# Autodesk Inventor assembly: GFRP_T2_03
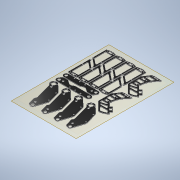
[picture p0: Inventor's stored thumbnail of the model, 180x180]
Saved by Autodesk Inventor 2022 (Build 260153000, 153)
## iProperties
Created: 2022-09-28
Part Number: GFRP_T2_03
Document SubType Name: Assembly
Designer: Masato
Author: Masato
## Documents named in this file (6)
- C:\Users\6343y\ドキュメント\Inventor\SUSTAINA-OP\Cam\GFRP_T2\OriginalMind_RD400\GFRP_T2_03.iam
- C:\Users\6343y\ドキュメント\Inventor\SUSTAINA-OP\Cam\DisposableBoard.ipt
- C:\Users\6343y\ドキュメント\Inventor\SUSTAINA-OP\LowerBody\Link\BackLink_frame.ipt
- C:\Users\6343y\ドキュメント\Inventor\SUSTAINA-OP\LowerBody\Link\FrontLink_frame.ipt
- C:\Users\6343y\ドキュメント\Inventor\SUSTAINA-OP\UpperBody\Arm\UpperArm_side_frame.ipt
- C:\Users\6343y\ドキュメント\Inventor\SUSTAINA-OP\UpperBody\Head\Head_neck_side_frame.ipt
## Components (17 placed, 5 different names)
1. DisposableBoard:1 — フラッシュ:1, フラッシュ:2, フラッシュ:3, フラッシュ:4, フラッシュ:9, フラッシュ:10, Tangent:23, Tangent:24
2. BackLink_frame:4 — メイト:21, Mate:25, Tangent:22
3. BackLink_frame:5 — Mate:24, Mate:25, Mate:26
4. UpperArm_side_frame:4 — フラッシュ:7, 正接:6, フラッシュ:10, メイト:15
5. UpperArm_side_frame:1 — メイト:12, フラッシュ:7, フラッシュ:9, 正接:6, Mate:26
6. UpperArm_side_frame:9
7. UpperArm_side_frame:10
8. UpperArm_side_frame:11
9. UpperArm_side_frame:12
10. UpperArm_side_frame:13 — Flush:11, Mate:23
11. UpperArm_side_frame:14
12. Head_neck_side_frame:1 — Mate:22, Flush:11, Mate:23
13. Head_neck_side_frame:2
14. FrontLink_frame:4 — メイト:13, Tangent:22, Tangent:23, Tangent:24
15. FrontLink_frame:5
16. FrontLink_frame:6
17. FrontLink_frame:7
## Component patterns: (4 elements, first: UpperArm_side_frame:4 + UpperArm_side_frame:1), (2 elements, first: Head_neck_side_frame:1), (4 elements, first: FrontLink_frame:4)
## Relationships (21: Mate 9, Flush 8, Tangent 4)
- フラッシュ:1 [Flush]: DisposableBoard:1
- フラッシュ:2 [Flush]: DisposableBoard:1
- フラッシュ:3 [Flush]: DisposableBoard:1
- フラッシュ:4 [Flush]: DisposableBoard:1
- メイト:12 [Mate]: UpperArm_side_frame:1
- フラッシュ:7 [Flush]: UpperArm_side_frame:4 ↔ UpperArm_side_frame:1
- フラッシュ:9 [Flush] (2 mm): DisposableBoard:1 ↔ UpperArm_side_frame:1
- 正接:6 [Tangent] (2.1 mm): UpperArm_side_frame:4 ↔ UpperArm_side_frame:1
- メイト:13 [Mate]: FrontLink_frame:4
- フラッシュ:10 [Flush] (-2.1 mm): DisposableBoard:1 ↔ UpperArm_side_frame:4
- メイト:15 [Mate]: UpperArm_side_frame:4
- メイト:21 [Mate]: BackLink_frame:4
- Mate:22: Head_neck_side_frame:1
- Flush:11: UpperArm_side_frame:13 ↔ Head_neck_side_frame:1
- Mate:23 (2.1 mm): UpperArm_side_frame:13 ↔ Head_neck_side_frame:1
- Mate:24: BackLink_frame:5
- Mate:25 (2.1 mm): BackLink_frame:4 ↔ BackLink_frame:5
- Mate:26 (2.1 mm): BackLink_frame:5 ↔ UpperArm_side_frame:1
- Tangent:22 (2.1 mm): BackLink_frame:4 ↔ FrontLink_frame:4
- Tangent:23 (2 mm): DisposableBoard:1 ↔ FrontLink_frame:4
- Tangent:24 (2 mm): DisposableBoard:1 ↔ FrontLink_frame:4
